# Autodesk Inventor assembly: Assembly
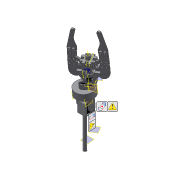
[picture p0: Inventor's stored thumbnail of the model, 180x180]
Saved by Autodesk Inventor 2018 (Build 220112000, 112)
## iProperties
Created: 2018-02-18
Part Number: Assembly
Document SubType Name: Assembly
Designer: Bardo91
Author: Bardo91
## Documents named in this file (11)
- E:\programming\hecatonquiros\cad_models\tools\gripper\serial_model_6DoF\Assembly.iam
- E:\programming\hecatonquiros\cad_models\tools\gripper\serial_model_6DoF\attachment.ipt
- E:\programming\hecatonquiros\cad_models\tools\gripper\serial_model_6DoF\microservo_FT.ipt
- E:\programming\hecatonquiros\cad_models\tools\gripper\serial_model_6DoF\base_gripper.ipt
- E:\programming\hecatonquiros\cad_models\tools\gripper\serial_model_6DoF\bar.ipt
- E:\programming\hecatonquiros\cad_models\tools\gripper\serial_model_6DoF\barMini.ipt
- E:\programming\hecatonquiros\cad_models\tools\gripper\serial_model_6DoF\holdBar.ipt
- E:\programming\hecatonquiros\cad_models\tools\gripper\serial_model_6DoF\gripper.ipt
- E:\programming\hecatonquiros\cad_models\tools\gripper\serial_model_6DoF\ScrewActuatorGripper.ipt
- E:\programming\hecatonquiros\cad_models\tools\gripper\serial_model_6DoF\ScrewActuatorGripperCenter.ipt
- E:\programming\hecatonquiros\cad_models\tools\gripper\serial_model_6DoF\middle_joint.ipt
## Components (22 placed, 10 different names)
1. attachment:1 — Mate:1, Mate:2, Mate:3, Mate:55
2. microservo_FT:1 — Mate:1, Mate:2, Mate:3, Mate:49, Flush:1, Mate:53
3. base_gripper:1 — Mate:5, Mate:6, Mate:7, Mate:8, Mate:9, Mate:10, Mate:11, Mate:12, Mate:13, Mate:49, Flush:1, Mate:50, Mate:51, Mate:52
4. microservo_FT:2 — Mate:5, Mate:6, Mate:7, Mate:40, Mate:41
5. bar:1 — Mate:27, Mate:28, Mate:44, Mate:47, Mate:60
6. bar:2 — Mate:29, Mate:30, Mate:59
7. bar:3 — Mate:31, Mate:34, Mate:56, Mate:61
8. bar:4 — Mate:32, Mate:33, Mate:58, Mate:59
9. bar:5 — Mate:14, Mate:15, Mate:64
10. bar:6 — Mate:16, Mate:17, Mate:57, Mate:63
11. bar:7 — Mate:18, Mate:19, Mate:65
12. bar:8 — Mate:20, Mate:21, Mate:43, Mate:46, Mate:62
13. barMini:1 — Mate:44, Mate:47, Mate:48, Mate:56
14. barMini:2 — Mate:43, Mate:45, Mate:46, Mate:57
15. holdBar:1 — Mate:11, Mate:12, Mate:13, Mate:14, Mate:15, Mate:16, Mate:17, Mate:18, Mate:19, Mate:20, Mate:21
16. holdBar:2 — Mate:8, Mate:9, Mate:10, Mate:27, Mate:28, Mate:29, Mate:30, Mate:31, Mate:32, Mate:33, Mate:34
17. ScrewActuatorGripper:1 — Mate:40, Mate:41, Mate:42
18. ScrewActuatorGripperCenter:1 — Mate:42, Mate:45, Mate:48
19. microservo_FT:3 — Mate:50, Mate:51, Mate:52, Mate:54, Mate:66
20. middle_joint:1 — Mate:53, Mate:54, Mate:55, Mate:66
21. gripper:1 — Mate:58, Mate:60, Mate:61
22. gripper:2 — Mate:62, Mate:63, Mate:64, Mate:65
## Relationships (56: Mate 55, Flush 1)
- Mate:1: attachment:1 ↔ microservo_FT:1
- Mate:2: attachment:1 ↔ microservo_FT:1
- Mate:3: attachment:1 ↔ microservo_FT:1
- Mate:5: base_gripper:1 ↔ microservo_FT:2
- Mate:6: base_gripper:1 ↔ microservo_FT:2
- Mate:7: base_gripper:1 ↔ microservo_FT:2
- Mate:8: base_gripper:1 ↔ holdBar:2
- Mate:9: base_gripper:1 ↔ holdBar:2
- Mate:10: base_gripper:1 ↔ holdBar:2
- Mate:11: base_gripper:1 ↔ holdBar:1
- Mate:12: base_gripper:1 ↔ holdBar:1
- Mate:13: base_gripper:1 ↔ holdBar:1
- Mate:14: bar:5 ↔ holdBar:1
- Mate:15: bar:5 ↔ holdBar:1
- Mate:16: bar:6 ↔ holdBar:1
- Mate:17: bar:6 ↔ holdBar:1
- Mate:18: bar:7 ↔ holdBar:1
- Mate:19: bar:7 ↔ holdBar:1
- Mate:20: bar:8 ↔ holdBar:1
- Mate:21: bar:8 ↔ holdBar:1
- Mate:27: bar:1 ↔ holdBar:2
- Mate:28: bar:1 ↔ holdBar:2
- Mate:29: bar:2 ↔ holdBar:2
- Mate:30: bar:2 ↔ holdBar:2
- Mate:31: bar:3 ↔ holdBar:2
- Mate:32: bar:4 ↔ holdBar:2
- Mate:33: bar:4 ↔ holdBar:2
- Mate:34: bar:3 ↔ holdBar:2
- Mate:40: microservo_FT:2 ↔ ScrewActuatorGripper:1
- Mate:41: microservo_FT:2 ↔ ScrewActuatorGripper:1
- Mate:42: ScrewActuatorGripper:1 ↔ ScrewActuatorGripperCenter:1
- Mate:43: bar:8 ↔ barMini:2
- Mate:44: bar:1 ↔ barMini:1
- Mate:45: barMini:2 ↔ ScrewActuatorGripperCenter:1
- Mate:46: bar:8 ↔ barMini:2
- Mate:47: bar:1 ↔ barMini:1
- Mate:48: barMini:1 ↔ ScrewActuatorGripperCenter:1
- Mate:49: microservo_FT:1 ↔ base_gripper:1
- Flush:1: microservo_FT:1 ↔ base_gripper:1
- Mate:50: base_gripper:1 ↔ microservo_FT:3
- Mate:51: base_gripper:1 ↔ microservo_FT:3
- Mate:52: base_gripper:1 ↔ microservo_FT:3
- Mate:53: microservo_FT:1 ↔ middle_joint:1
- Mate:54: microservo_FT:3 ↔ middle_joint:1
- Mate:55 (0.5 mm): attachment:1 ↔ middle_joint:1
- Mate:56: bar:3 ↔ barMini:1
- Mate:57: bar:6 ↔ barMini:2
- Mate:58: bar:4 ↔ gripper:1
- Mate:59: bar:2 ↔ bar:4
- Mate:60: bar:1 ↔ gripper:1
- Mate:61: bar:3 ↔ gripper:1
- Mate:62: bar:8 ↔ gripper:2
- Mate:63: bar:6 ↔ gripper:2
- Mate:64: bar:5 ↔ gripper:2
- Mate:65: bar:7 ↔ gripper:2
- Mate:66: microservo_FT:3 ↔ middle_joint:1
